# Autodesk Inventor assembly: dads real trunk assembly
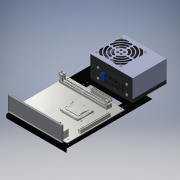
[picture p0: Inventor's stored thumbnail of the model, 180x180]
Saved by Autodesk Inventor 2018 (Build 220112000, 112)
## iProperties
Created: 2018-06-20
Part Number: dads real trunk assembly
Document SubType Name: Assembly
Designer: John Viljoen
Author: John Viljoen
## Documents named in this file (6)
- C:\Users\John Viljoen\Documents\Inventor\computer project\dads real trunk assembly.iam
- C:\Users\John Viljoen\Documents\Inventor\computer project\dads real trunk.ipt
- C:\Users\John Viljoen\Documents\Inventor\computer project\Mini-ITX Mobo.ipt
- C:\Users\John Viljoen\Documents\Inventor\computer project\io_shield.ipt
- C:\Users\John Viljoen\Documents\Inventor\computer project\sfx psu from grabCAD\sfx 45g.iam
- C:\Users\John Viljoen\Documents\Inventor\computer project\psu mount.ipt
## Components (5 placed, 5 different names)
1. dads real trunk:1 — Flush:1, Flush:2, Mate:1, Mate:5
2. Mini-ITX Mobo:1 — Flush:1, Flush:2, Mate:1, Mate:2, Mate:3, Mate:4, Mate:6, Flush:3
3. io_shield:1 — Mate:2, Mate:3, Mate:4
4. sfx 45g:1 [sub-assembly] — Mate:5, Mate:6, Flush:3, Mate:7, Flush:4, Flush:5
5. psu mount:1 — Mate:7, Flush:4, Flush:5
## Relationships (12: Mate 7, Flush 5)
- Flush:1 (5.677 mm): dads real trunk:1 ↔ Mini-ITX Mobo:1
- Flush:2 (3.82 mm): dads real trunk:1 ↔ Mini-ITX Mobo:1
- Mate:1 (10 mm): dads real trunk:1 ↔ Mini-ITX Mobo:1
- Mate:2 (1 mm): Mini-ITX Mobo:1 ↔ io_shield:1
- Mate:3: Mini-ITX Mobo:1 ↔ io_shield:1
- Mate:4 (1 mm): Mini-ITX Mobo:1 ↔ io_shield:1
- Mate:5: dads real trunk:1 ↔ sfx 45g:1
- Mate:6 (40 mm): Mini-ITX Mobo:1 ↔ sfx 45g:1
- Flush:3 (-5 mm): Mini-ITX Mobo:1 ↔ sfx 45g:1
- Mate:7: sfx 45g:1 ↔ psu mount:1
- Flush:4 (0.5 mm): sfx 45g:1 ↔ psu mount:1
- Flush:5: sfx 45g:1 ↔ psu mount:1
